# Autodesk Inventor assembly: garra2
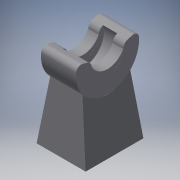
[picture p0: Inventor's stored thumbnail of the model, 180x180]
Saved by Autodesk Inventor 2018 (Build 220112000, 112)
## iProperties
Created: 2020-01-23
Part Number: garra2
Document SubType Name: Assembly
Designer: peter
Author: peter
## Documents named in this file (4)
- C:\Users\peter\Desktop\INGENIERIA USAC\INVENTOR3D\SmartCar\garra2.iam
- C:\Users\peter\Desktop\INGENIERIA USAC\INVENTOR3D\SmartCar\BaseGarra.ipt
- C:\Users\peter\Desktop\INGENIERIA USAC\INVENTOR3D\SmartCar\GarraBearing.ipt
- C:\Users\peter\Desktop\INGENIERIA USAC\INVENTOR3D\SmartCar\Tapa.ipt
## Components (4 placed, 3 different names)
1. BaseGarra:1 — Mate:1
2. GarraBearing:1 — Mate:1, Mate:2, Flush:1, Flush:2
3. Tapa:1 — Flush:2
4. Tapa:2 — Mate:2, Flush:1
## Relationships (4: Mate 2, Flush 2)
- Mate:1: BaseGarra:1 ↔ GarraBearing:1
- Mate:2: GarraBearing:1 ↔ Tapa:2
- Flush:1: GarraBearing:1 ↔ Tapa:2
- Flush:2: GarraBearing:1 ↔ Tapa:1
